# Autodesk Inventor assembly: lod assy
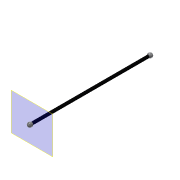
[picture p0: Inventor's stored thumbnail of the model, 180x180]
Saved by Autodesk Inventor 2016 (Build 200138000, 138)
## iProperties
Created: 2016-08-18
Part Number: lod assy
Document SubType Name: Assembly
Designer: admin
Author: admin
## Documents named in this file (3)
- H:\Ateam ventures\creatablaeD3\최종 3D 도면 0818\lod assy\lod assy.iam
- H:\Ateam ventures\creatablaeD3\최종 3D 도면 0818\lod assy\ball_tap.ipt
- H:\Ateam ventures\creatablaeD3\최종 3D 도면 0818\lod assy\rod.ipt
## Components (3 placed, 2 different names)
1. ball_tap:1 — Rotational:3
2. rod:1 — Rotational:2, Rotational:3
3. ball_tap:2 — Rotational:2
## Relationships (2: RevoluteJoint 2)
- Rotational:2 [RevoluteJoint]: rod:1 ↔ ball_tap:2
- Rotational:3 [RevoluteJoint]: ball_tap:1 ↔ rod:1
